# Autodesk Inventor assembly: VolteraOne_tool.ipj
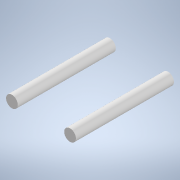
[picture p0: Inventor's stored thumbnail of the model, 180x180]
Saved by Autodesk Inventor 2022 (Build 260153000, 153)
## iProperties
Created: 2022-08-22
Part Number: VolteraOne_tool.ipj
Document SubType Name: Assembly
Designer: diederichbenedict
Author: diederichbenedict
## Documents named in this file (2)
- C:\Users\diederichbenedict\Dropbox\Dokumente\Promotion\PROJECTS\VOLTERA\INVENTOR\VolteraOne_tool.ipj.iam
- C:\Users\diederichbenedict\Dropbox\Dokumente\Promotion\PROJECTS\VOLTERA\INVENTOR\00_rod_6mm.ipt
## Components (2 placed, 1 different names)
1. 00_rod_6mm:1
2. 00_rod_6mm:2
## Component patterns: (2 elements, first: 00_rod_6mm:1)
